# Autodesk Inventor assembly: SimplifiedLeg
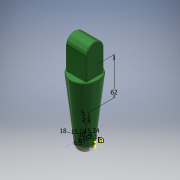
[picture p0: Inventor's stored thumbnail of the model, 180x180]
Saved by Autodesk Inventor 2018 (Build 220112000, 112)
## iProperties
Part Number: SimplifiedLeg
Material: Generisch
Document SubType Name: Assembly
Designer: Jochen Alt
Mass: 279.988 g
Surface Area: 1394.51 cm^2
Volume: 279.988 cm^3
Density: 1 g/cm^3
Author: Jochen Alt
## Documents named in this file (6)
- D:\Projects\Manfred\cad\Inventor\SimplifiedLeg.iam
- D:\Projects\Manfred\cad\Inventor\Hip.ipt
- E:\Projects\Manfred\cad\simplified\DrehAchse.ipt
- D:\Projects\Manfred\cad\Inventor\HipJoint.ipt
- D:\Projects\Manfred\cad\Inventor\Thigh.ipt
- D:\Projects\Manfred\cad\simplified\SimplifiedFoot.ipt
## Components (5 placed, 5 different names)
1. Hip:1 — Winkel:1, Passend:1, Fluchtend:1
2. HipJoint:1 — Passend:3, Passend:4, Winkel:3
3. Thigh:1 — Passend:2, Fluchtend:2, Winkel:2
4. DrehAchse:1 — Passend:1, Fluchtend:1, Passend:2, Fluchtend:2, Passend:3, Passend:4, Passend:5, Winkel:4, Passend:6
5. SimplifiedFoot:1 — Passend:5, Winkel:4, Passend:6
## Relationships (12: Mate 6, Angle 4, Flush 2)
- Winkel:1 [Angle] (0 deg): Hip:1
- Passend:1 [Mate]: Hip:1 ↔ DrehAchse:1
- Fluchtend:1 [Flush]: Hip:1 ↔ DrehAchse:1
- Passend:2 [Mate]: Thigh:1 ↔ DrehAchse:1
- Fluchtend:2 [Flush]: Thigh:1 ↔ DrehAchse:1
- Winkel:2 [Angle] (0 deg): Thigh:1
- Passend:3 [Mate]: HipJoint:1 ↔ DrehAchse:1
- Passend:4 [Mate] (1 mm): HipJoint:1 ↔ DrehAchse:1
- Winkel:3 [Angle] (0 deg): HipJoint:1
- Passend:5 [Mate]: DrehAchse:1 ↔ SimplifiedFoot:1
- Winkel:4 [Angle] (0 deg): DrehAchse:1 ↔ SimplifiedFoot:1
- Passend:6 [Mate]: DrehAchse:1 ↔ SimplifiedFoot:1
